# Autodesk Inventor assembly: Drumstick
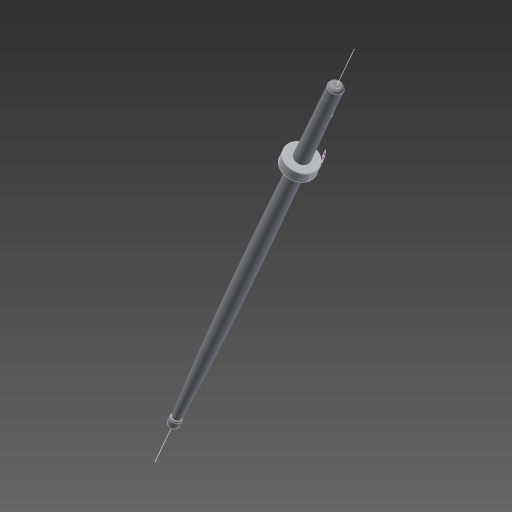
[picture p0: Inventor's stored thumbnail of the model, 512x512]
Saved by Autodesk Inventor 2023 (Build 270158000, 158)
## iProperties
Created: 2020-03-24
Part Number: Drumstick
Document SubType Name: Assembly
Designer: valer
Mass: 4853.13 g
Surface Area: 3141.52 cm^2
Volume: 1403.99 cm^3
Density: 3.45667 g/cm^3
Author: valer
## Documents named in this file (4)
- C:\Users\Val\Desktop\str1ker\parts\Drumstick.iam
- C:\Users\Val\Desktop\str1ker\parts\external\Drumstick.ipt
- C:\Users\Val\Desktop\str1ker\parts\external\ForearmShaftCollar.ipt
- C:\Users\Val\Desktop\str1ker\description\models\src\DrumstickBoundingBox.ipt
## Components (3 placed, 3 different names)
1. Drumstick:1 — Mate:79, Flush:3, Angle:1
2. ShaftCollar1/2:1 — Mate:79, Flush:3, Mate:81, Flush:4
3. DrumstickBoundingBox:1 — Flush:5, Flush:6, Flush:7, Mate:82
## Relationships (9: Flush 5, Mate 3, Angle 1)
- Mate:79: Drumstick:1 ↔ ShaftCollar1/2:1
- Flush:3 (304.8 mm): Drumstick:1 ↔ ShaftCollar1/2:1
- Mate:81: ShaftCollar1/2:1
- Flush:4: ShaftCollar1/2:1
- Flush:5: DrumstickBoundingBox:1
- Angle:1 (180 deg): Drumstick:1
- Flush:6: DrumstickBoundingBox:1
- Flush:7: DrumstickBoundingBox:1
- Mate:82: DrumstickBoundingBox:1
